# Autodesk Inventor assembly: Case-ASMB
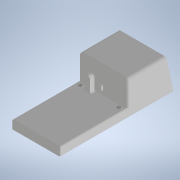
[picture p0: Inventor's stored thumbnail of the model, 180x180]
Saved by Autodesk Inventor 2022 (Build 260153000, 153)
## iProperties
Created: 2023-12-02
Part Number: Case-ASMB
Document SubType Name: Assembly
Designer: Egor
Author: Egor
## Documents named in this file (7)
- C:\Study\Artemiev\case\Case-ASMB.iam
- C:\Study\Artemiev\case\Base.ipt
- C:\Study\Artemiev\case\pcb\PCB1.iam
- C:\Study\Artemiev\case\Cap.ipt
- C:\Study\Artemiev\case\Втулка_2.ipt
- C:\Users\user\Documents\Inventor\Content Center Files\R2022\ru-RU\BS EN ISO 7045 Z\EN ISO 7045 - M3 x 5 - 4.8 - Z(1).ipt
- C:\Study\Artemiev\case\Temp_Module.ipt
## Components (24 placed, 6 different names)
1. Base:1 — С поворотом:1, С поворотом:2, Insert:1, Insert:2, Insert:3, Insert:4, Insert:5, Insert:15, Insert:16, Insert:17, Insert:18, Insert:19, Insert:20
2. PCB1:1 [sub-assembly] — С поворотом:1, Insert:10, Insert:20, Insert:21, Insert:22, Insert:23, Insert:24
3. Cap:1 — С поворотом:2, Insert:6, Insert:7, Insert:8, Insert:9, Insert:15, Mate:5, Mate:6
4. Втулка_2:1 — Insert:3
5. Втулка_2:2 — Insert:1
6. Втулка_2:3 — Insert:2
7. Втулка_2:4 — Insert:21
8. Втулка_2:5 — Insert:4, Mate:4
9. Втулка_2:6 — Insert:5, Insert:12
10. Втулка_2:7 — Insert:9
11. Втулка_2:8 — Insert:8
12. Втулка_2:9 — Insert:7
13. Втулка_2:10 — Insert:6
14. BS EN ISO 7045 Z - метрическая M3 x 5 - 4.8 - Z:1 — Insert:10
15. BS EN ISO 7045 Z - метрическая M3 x 5 - 4.8 - Z:2 — Insert:24
16. BS EN ISO 7045 Z - метрическая M3 x 5 - 4.8 - Z:3 — Insert:22
17. BS EN ISO 7045 Z - метрическая M3 x 5 - 4.8 - Z:4 — Insert:23
18. BS EN ISO 7045 Z - метрическая M3 x 5 - 4.8 - Z:5 — Insert:13
19. BS EN ISO 7045 Z - метрическая M3 x 5 - 4.8 - Z:6 — Insert:14
20. BS EN ISO 7045 Z - метрическая M3 x 5 - 4.8 - Z:7 — Insert:16
21. BS EN ISO 7045 Z - метрическая M3 x 5 - 4.8 - Z:8 — Insert:17
22. BS EN ISO 7045 Z - метрическая M3 x 5 - 4.8 - Z:9 — Insert:18
23. BS EN ISO 7045 Z - метрическая M3 x 5 - 4.8 - Z:10 — Insert:19
24. Temp_Module:1 — Insert:12, Mate:4, Insert:13, Insert:14
## Relationships (28: Insert 23, Mate 3, RevoluteJoint 2)
- С поворотом:1 [RevoluteJoint]: Base:1 ↔ PCB1:1
- С поворотом:2 [RevoluteJoint]: Base:1 ↔ Cap:1
- Insert:1: Base:1 ↔ Втулка_2:2
- Insert:2: Base:1 ↔ Втулка_2:3
- Insert:3: Base:1 ↔ Втулка_2:1
- Insert:4: Base:1 ↔ Втулка_2:5
- Insert:5: Base:1 ↔ Втулка_2:6
- Insert:6: Cap:1 ↔ Втулка_2:10
- Insert:7: Cap:1 ↔ Втулка_2:9
- Insert:8: Cap:1 ↔ Втулка_2:8
- Insert:9: Cap:1 ↔ Втулка_2:7
- Insert:10: PCB1:1 ↔ BS EN ISO 7045 Z - метрическая M3 x 5 - 4.8 - Z:1
- Insert:12: Втулка_2:6 ↔ Temp_Module:1
- Mate:4: Втулка_2:5 ↔ Temp_Module:1
- Insert:13: BS EN ISO 7045 Z - метрическая M3 x 5 - 4.8 - Z:5 ↔ Temp_Module:1
- Insert:14: BS EN ISO 7045 Z - метрическая M3 x 5 - 4.8 - Z:6 ↔ Temp_Module:1
- Insert:15: Base:1 ↔ Cap:1
- Insert:16: Base:1 ↔ BS EN ISO 7045 Z - метрическая M3 x 5 - 4.8 - Z:7
- Insert:17: Base:1 ↔ BS EN ISO 7045 Z - метрическая M3 x 5 - 4.8 - Z:8
- Insert:18: Base:1 ↔ BS EN ISO 7045 Z - метрическая M3 x 5 - 4.8 - Z:9
- Insert:19: Base:1 ↔ BS EN ISO 7045 Z - метрическая M3 x 5 - 4.8 - Z:10
- Mate:5: Cap:1
- Mate:6: Cap:1
- Insert:20: Base:1 ↔ PCB1:1
- Insert:21: PCB1:1 ↔ Втулка_2:4
- Insert:22: PCB1:1 ↔ BS EN ISO 7045 Z - метрическая M3 x 5 - 4.8 - Z:3
- Insert:23: PCB1:1 ↔ BS EN ISO 7045 Z - метрическая M3 x 5 - 4.8 - Z:4
- Insert:24: PCB1:1 ↔ BS EN ISO 7045 Z - метрическая M3 x 5 - 4.8 - Z:2
